# Autodesk Inventor assembly: demo_finley_gripper
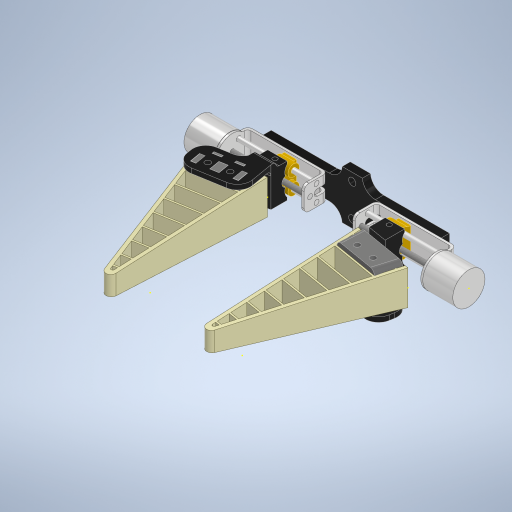
[picture p0: Inventor's stored thumbnail of the model, 512x512]
Saved by Autodesk Inventor 2024 (Build 280153000, 153)
## iProperties
Created: 2024-10-06
Part Number: demo_finley_gripper
Document SubType Name: Assembly
Designer: 1412z
Author: 1412z
## Documents named in this file (10)
- C:\Users\1412z\OneDrive\デスクトップ\rdclab\harvesting_robot\harvesting_endeffector\demo_finley_gripper\demo_finley_gripper.iam
- C:\Users\1412z\OneDrive\デスクトップ\rdclab\harvesting_robot\harvesting_endeffector\finley_gripper\fixed_parts\base.ipt
- C:\Users\1412z\OneDrive\デスクトップ\rdclab\harvesting_robot\harvesting_endeffector\linear_slider\body.ipt
- C:\Users\1412z\OneDrive\デスクトップ\rdclab\harvesting_robot\harvesting_endeffector\linear_slider\stepping_motor.ipt
- C:\Users\1412z\OneDrive\デスクトップ\rdclab\harvesting_robot\harvesting_endeffector\linear_slider\shaft_screw.ipt
- C:\Users\1412z\OneDrive\デスクトップ\rdclab\harvesting_robot\harvesting_endeffector\linear_slider\shaft.ipt
- C:\Users\1412z\OneDrive\デスクトップ\rdclab\harvesting_robot\harvesting_endeffector\linear_slider\moving_part.ipt
- C:\Users\1412z\OneDrive\デスクトップ\rdclab\harvesting_robot\harvesting_endeffector\finley_gripper\fixed_parts\finlay_holds_board.ipt
- C:\Users\1412z\OneDrive\デスクトップ\rdclab\harvesting_robot\harvesting_endeffector\finley_gripper\fixed_parts\finlay_holds_down.ipt
- C:\Users\1412z\OneDrive\デスクトップ\rdclab\harvesting_robot\harvesting_endeffector\finley_gripper\finley_gripper_80.ipt
## Components (19 placed, 9 different names)
1. base:1 — 回転:1, 回転:2, 回転:3, 回転:4
2. body:1 — 回転:1, 回転:2, メイト:1, メイト:2, メイト:3, メイト:9, メイト:15, メイト:17, メイト:18
3. body:2 — 回転:3, 回転:4, メイト:4, メイト:5, メイト:6, メイト:7, メイト:8, メイト:11, メイト:13
4. stepping_motor:1 — メイト:1, メイト:2, メイト:3, メイト:10, メイト:16
5. stepping_motor:2 — メイト:4, メイト:5, メイト:6, メイト:12, メイト:14
6. shaft_screw:1 — メイト:7, メイト:8
7. shaft_screw:2 — メイト:9, メイト:10
8. shaft:1 — メイト:13, メイト:14, 円柱状:4
9. shaft:2 — メイト:11, メイト:12, 円柱状:3
10. shaft:3 — メイト:17, メイト:18, 円柱状:2
11. shaft:4 — メイト:15, メイト:16, 円柱状:1
12. moving_part:1 — 円柱状:3, 円柱状:4, 挿入:1
13. moving_part:2 — 円柱状:1, 円柱状:2, 挿入:2
14. finlay_holds_board:1 — 挿入:1, 円柱状:7, 円柱状:8
15. finlay_holds_board:2 — 挿入:2, 円柱状:5, 円柱状:6
16. finlay_holds_down:1 — 円柱状:7, 円柱状:8, メイト:20
17. finlay_holds_down:2 — 円柱状:5, 円柱状:6, メイト:19
18. finley_gripper_80:1 — メイト:19
19. finley_gripper_80:2 — メイト:20
## Relationships (34: Mate 20, CylindricalJoint 8, RevoluteJoint 4, Insert 2)
- 回転:1 [RevoluteJoint]: base:1 ↔ body:1
- 回転:2 [RevoluteJoint]: base:1 ↔ body:1
- 回転:3 [RevoluteJoint]: base:1 ↔ body:2
- 回転:4 [RevoluteJoint]: base:1 ↔ body:2
- メイト:1 [Mate]: body:1 ↔ stepping_motor:1
- メイト:2 [Mate]: body:1 ↔ stepping_motor:1
- メイト:3 [Mate]: body:1 ↔ stepping_motor:1
- メイト:4 [Mate]: body:2 ↔ stepping_motor:2
- メイト:5 [Mate]: body:2 ↔ stepping_motor:2
- メイト:6 [Mate]: body:2 ↔ stepping_motor:2
- メイト:7 [Mate]: body:2 ↔ shaft_screw:1
- メイト:8 [Mate]: body:2 ↔ shaft_screw:1
- メイト:9 [Mate]: body:1 ↔ shaft_screw:2
- メイト:10 [Mate]: stepping_motor:1 ↔ shaft_screw:2
- メイト:11 [Mate]: body:2 ↔ shaft:2
- メイト:12 [Mate]: stepping_motor:2 ↔ shaft:2
- メイト:13 [Mate]: body:2 ↔ shaft:1
- メイト:14 [Mate]: stepping_motor:2 ↔ shaft:1
- メイト:15 [Mate]: body:1 ↔ shaft:4
- メイト:16 [Mate]: stepping_motor:1 ↔ shaft:4
- メイト:17 [Mate]: body:1 ↔ shaft:3
- メイト:18 [Mate]: body:1 ↔ shaft:3
- 円柱状:1 [CylindricalJoint]: shaft:4 ↔ moving_part:2
- 円柱状:2 [CylindricalJoint]: shaft:3 ↔ moving_part:2
- 円柱状:3 [CylindricalJoint]: shaft:2 ↔ moving_part:1
- 円柱状:4 [CylindricalJoint]: shaft:1 ↔ moving_part:1
- 挿入:1 [Insert]: moving_part:1 ↔ finlay_holds_board:1
- 挿入:2 [Insert]: moving_part:2 ↔ finlay_holds_board:2
- 円柱状:5 [CylindricalJoint]: finlay_holds_board:2 ↔ finlay_holds_down:2
- 円柱状:6 [CylindricalJoint]: finlay_holds_board:2 ↔ finlay_holds_down:2
- 円柱状:7 [CylindricalJoint]: finlay_holds_board:1 ↔ finlay_holds_down:1
- 円柱状:8 [CylindricalJoint]: finlay_holds_board:1 ↔ finlay_holds_down:1
- メイト:19 [Mate] (-10.8 mm): finlay_holds_down:2 ↔ finley_gripper_80:1
- メイト:20 [Mate] (-10.8 mm): finlay_holds_down:1 ↔ finley_gripper_80:2
